# Autodesk Inventor assembly: AirtightAftSectionAssembly0
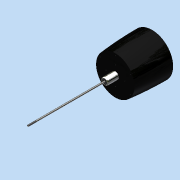
[picture p0: Inventor's stored thumbnail of the model, 180x180]
Saved by Autodesk Inventor 2017 (Build 210142000, 142)
## iProperties
Created: 2016-10-23
Part Number: AirtightAftSectionAssembly0
Document SubType Name: Assembly
Designer: techn
Author: techn
## Documents named in this file (6)
- D:\OneDrive\Documents\Other Projects\Submarine\CAD\aft\AirtightAftSectionAssembly0.iam
- D:\OneDrive\Documents\Other Projects\Submarine\CAD\aft\MotorAssembly0.iam
- D:\OneDrive\Documents\Other Projects\Submarine\CAD\aft\AftSectionAirtightRear.ipt
- D:\OneDrive\Documents\Other Projects\Submarine\CAD\aft\ServoAssembly\aftServoAssemblyForwardDisc.ipt
- D:\OneDrive\Documents\Other Projects\Submarine\CAD\common\HitecServo\HitecServoAssembly.iam
- D:\OneDrive\Documents\Other Projects\Submarine\CAD\aft\ServoAssembly\aftServoAssemblyFrontDisc.ipt
## Components (6 placed, 5 different names)
1. MotorAssembly0:1 [sub-assembly] — Mate:5, Mate:6, Mate:7, Mate:8
2. AftSectionAirtightRear:1 — Mate:5, Mate:6, Mate:7, Mate:9, Mate:10
3. aftServoAssemblyForwardDisc:1 — Mate:1, Mate:2, Mate:3, Mate:4, Angle:1, Angle:2, Mate:8, Mate:9, Mate:10
4. HitecServoAssembly:1 [sub-assembly] — Mate:2, Mate:3, Angle:1, Mate:12
5. HitecServoAssembly:2 [sub-assembly] — Mate:1, Mate:4, Angle:2, Mate:11, Mate:13
6. aftServoAssemblyFrontDisc:1 — Mate:11, Mate:12, Mate:13
## Relationships (15: Mate 13, Angle 2)
- Mate:1: aftServoAssemblyForwardDisc:1 ↔ HitecServoAssembly:2
- Mate:2: aftServoAssemblyForwardDisc:1 ↔ HitecServoAssembly:1
- Mate:3: aftServoAssemblyForwardDisc:1 ↔ HitecServoAssembly:1
- Mate:4: aftServoAssemblyForwardDisc:1 ↔ HitecServoAssembly:2
- Angle:1 (0 deg): aftServoAssemblyForwardDisc:1 ↔ HitecServoAssembly:1
- Angle:2 (0 deg): aftServoAssemblyForwardDisc:1 ↔ HitecServoAssembly:2
- Mate:5: MotorAssembly0:1 ↔ AftSectionAirtightRear:1
- Mate:6: MotorAssembly0:1 ↔ AftSectionAirtightRear:1
- Mate:7: MotorAssembly0:1 ↔ AftSectionAirtightRear:1
- Mate:8: MotorAssembly0:1 ↔ aftServoAssemblyForwardDisc:1
- Mate:9: AftSectionAirtightRear:1 ↔ aftServoAssemblyForwardDisc:1
- Mate:10 (15.875 mm): AftSectionAirtightRear:1 ↔ aftServoAssemblyForwardDisc:1
- Mate:11: HitecServoAssembly:2 ↔ aftServoAssemblyFrontDisc:1
- Mate:12: HitecServoAssembly:1 ↔ aftServoAssemblyFrontDisc:1
- Mate:13: HitecServoAssembly:2 ↔ aftServoAssemblyFrontDisc:1
